# Autodesk Inventor assembly: Assembly2
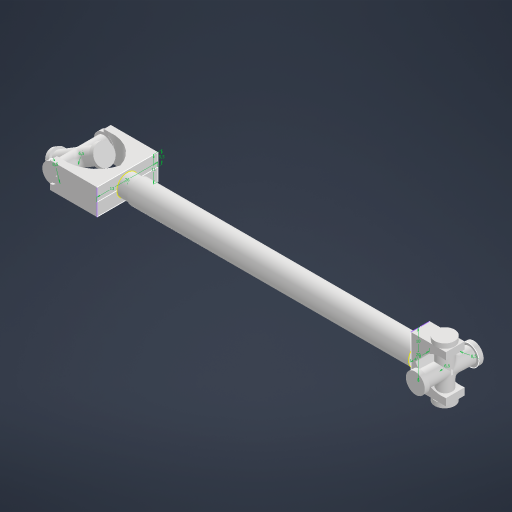
[picture p0: Inventor's stored thumbnail of the model, 512x512]
Saved by Autodesk Inventor 2023 (Build 270158030, 158C)
## iProperties
Created: 2023-02-03
Part Number: Assembly2
Document SubType Name: Assembly
Designer: Monster
Author: Monster
## Documents named in this file (3)
- C:\Users\Monster\Desktop\Ders\UKA\shaft\Assembly2.iam
- C:\Users\Monster\Desktop\Ders\UKA\shaft\Part1.ipt
- C:\Users\Monster\Desktop\Ders\UKA\shaft\Part2.ipt
## Components (3 placed, 2 different names)
1. Part1:1 — Mate:1, Mate:2, Mate:3, Mate:4
2. Part2:1 — Mate:1, Mate:2
3. Part2:2 — Mate:3, Mate:4
## Relationships (4: Mate 4)
- Mate:1: Part1:1 ↔ Part2:1
- Mate:2: Part1:1 ↔ Part2:1
- Mate:3: Part1:1 ↔ Part2:2
- Mate:4 (1 mm): Part1:1 ↔ Part2:2
